# Autodesk Inventor assembly: guidage_lineaire_shs55_lv_1_ss___492l_66
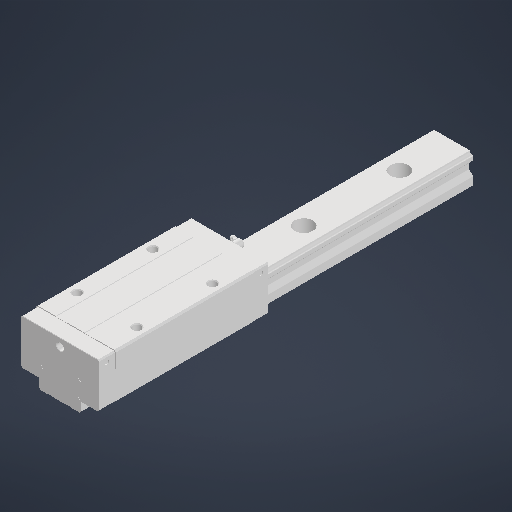
[picture p0: Inventor's stored thumbnail of the model, 512x512]
Saved by Autodesk Inventor 2025 (Build 290162000, 162)
## iProperties
Company: TraceParts S.A.
Created: 2024-05-27
Part Number: guidage_lineaire_shs55_lv_1_ss___492l_66
Checked By: TraceParts S.A.
Catalog Web Link: www.traceparts.com
Document SubType Name: Assembly
Designer: TraceParts
Sending System: TraceParts v2
Major Version: 6.0
Minor Version: 0.0
Format Version: 0.0
Product Id: TraceParts v2
REFERENCE: SHS55 LV 1 SS + 492L
SUPPLIER: THK
DESIGN: Linear guide SHS55LV type, 1 block(s), Without QZ lubricator, SS - With end, side, inner seals, Preload type: normal clearance, Rail length: 492 mm, Accuracy grade: Normal grade, Symmetric G dimension: G=66mm
MASS: 12.364
TraceParts.PartNumber: 10-08102015-095416
TraceParts.PartVersion: 1.1.3
TraceParts.InstanceId: 10-08102015-0954164NJ7PXS09GQEYYQMYO75F4N7R
TraceParts.PartTitle: Caged Ball LM Guide Global Standard Size Model SHS-LV
TRACEPARTS: TRACEPARTS
TraceParts.PartLanguage: en
Author: TraceParts
## Documents named in this file (3)
- D:\UNAL\2024-1S\APM\Digital Factory\Linear Guides & Ball Screws\guidage_lineaire_shs55_lv_1_ss___492l_66.iam
- D:\UNAL\2024-1S\APM\Digital Factory\Linear Guides & Ball Screws\guidage_lineaire_shs55_lv_1_ss___492l_66_01.ipt
- D:\UNAL\2024-1S\APM\Digital Factory\Linear Guides & Ball Screws\guidage_lineaire_shs55_lv_1_ss___492l_66_02.ipt
## Components (2 placed, 2 different names)
1. guidage_lineaire_shs55_lv_1_ss___492l_66_Temp_1:1 — Slider:1
2. guidage_lineaire_shs55_lv_1_ss___492l_66_Temp_2:1 — Slider:1
## Relationships (1: TranslationJoint 1)
- Slider:1 [TranslationJoint]: guidage_lineaire_shs55_lv_1_ss___492l_66_Temp_1:1 ↔ guidage_lineaire_shs55_lv_1_ss___492l_66_Temp_2:1
